# Autodesk Inventor assembly: ASY NDM 11.037 упор
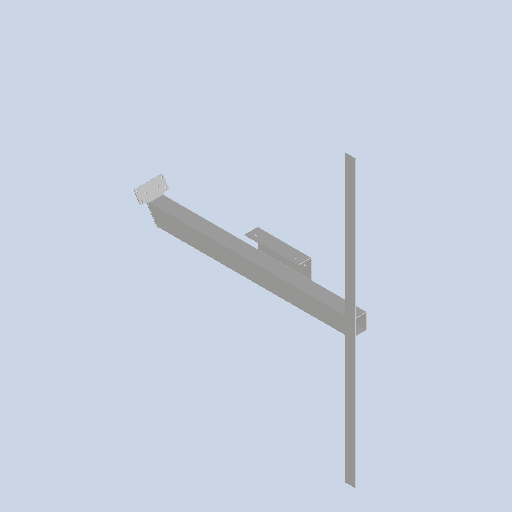
[picture p0: Inventor's stored thumbnail of the model, 512x512]
Saved by Autodesk Inventor 2025 (Build 290162010, 162A)
## iProperties
Created: 2024-08-18
Part Number: ASY NDM 11.037 упор
Document SubType Name: Assembly
Designer: admin
Author: admin
## Documents named in this file (5)
- C:\Users\pokla\Documents\Inventor\BSH_Beshkino_bio_tank\лестница\Перегородка\ASY NDM 11.037 упор.iam
- C:\Users\pokla\Documents\Inventor\BSH_Beshkino_bio_tank\лестница\Перегородка\NDM 11.034 упор.ipt
- C:\Users\pokla\Documents\Inventor\BSH_Beshkino_bio_tank\Trommel separator old\Part2.ipt
- C:\Users\pokla\Documents\Inventor\BSH_Beshkino_bio_tank\лестница\кронштейн\NDM 11.046 кронштейн .ipt
- C:\Users\pokla\Documents\Inventor\BSH_Beshkino_bio_tank\лестница\кронштейн\NDM 11.047 пластина.ipt
## Components (4 placed, 4 different names)
1. NDM 11.034 упор:1 — Mate:3, Mate:4, Rigid:1
2. Part2:1
3. NDM 11.046 кронштейн :1 — Mate:3, Mate:4
4. NDM 11.047 пластина:1 — Rigid:1
## Relationships (7: Mate 4, Flush 2, WeldJoint 1)
- [Flush]: NDM 11.034 упор:1 ↔ Part2:1
- [Mate]: NDM 11.034 упор:1 ↔ Part2:1
- [Flush]: NDM 11.034 упор:1 ↔ Part2:1
- [Mate]: NDM 11.034 упор:1 ↔ Part2:1
- Mate:3: NDM 11.034 упор:1 ↔ NDM 11.046 кронштейн :1
- Mate:4: NDM 11.034 упор:1 ↔ NDM 11.046 кронштейн :1
- Rigid:1 [WeldJoint]: NDM 11.034 упор:1 ↔ NDM 11.047 пластина:1
